# Autodesk Inventor assembly: DarkPoolFacility
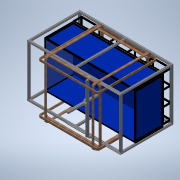
[picture p0: Inventor's stored thumbnail of the model, 180x180]
Saved by Autodesk Inventor 2022 (Build 260153000, 153)
## iProperties
Created: 2021-05-11
Part Number: DarkPoolFacility
Document SubType Name: Assembly
Designer: jamieson-bl
Author: jamieson-bl
## Documents named in this file (9)
- \\Mac\Home\Desktop\WinnipegPMTTestFacility\DarkPoolFacility.iam
- \\Mac\Home\Desktop\WinnipegPMTTestFacility\Room3L10.ipt
- \\Mac\Home\Desktop\WinnipegPMTTestFacility\iManikins\iMan\iMan.iam
- \\Mac\Home\Desktop\WinnipegPMTTestFacility\iManikins\iMandy\iMandy.iam
- \\Mac\Home\Desktop\WinnipegPMTTestFacility\Field Compensation Coils.iam
- \\Mac\Home\Desktop\WinnipegPMTTestFacility\ElectronicsRack.ipt
- \\Mac\Home\Desktop\WinnipegPMTTestFacility\CustomAquariumsStand.ipt
- \\Mac\Home\Desktop\WinnipegPMTTestFacility\CustomAquariumsTank.ipt
- \\Mac\Home\Desktop\WinnipegPMTTestFacility\gantry design\6060gantry.iam
## Components (8 placed, 8 different names)
1. Room3L10:1 — Mate:2, Mate:3
2. iMan:1 [sub-assembly] — Mate:3
3. iMandy:1 [sub-assembly] — Mate:2
4. Field Compensation Coils:1 [sub-assembly] — Mate:5, Mate:6, Mate:7
5. ElectronicsRack:1
6. CustomAquariumsStand:1 — Mate:4, Flush:1, Flush:2, Mate:5, Mate:6, Flush:3, Mate:9
7. CustomAquariumsTank:1 — Mate:4, Flush:1, Flush:2, Mate:7, Mate:8
8. 6060gantry:1 [sub-assembly] — Flush:3, Mate:8, Mate:9
## Relationships (11: Mate 8, Flush 3)
- Mate:2: Room3L10:1 ↔ iMandy:1
- Mate:3: Room3L10:1 ↔ iMan:1
- Mate:4: CustomAquariumsStand:1 ↔ CustomAquariumsTank:1
- Flush:1: CustomAquariumsStand:1 ↔ CustomAquariumsTank:1
- Flush:2: CustomAquariumsStand:1 ↔ CustomAquariumsTank:1
- Mate:5: Field Compensation Coils:1 ↔ CustomAquariumsStand:1
- Mate:6: Field Compensation Coils:1 ↔ CustomAquariumsStand:1
- Mate:7: Field Compensation Coils:1 ↔ CustomAquariumsTank:1
- Flush:3: CustomAquariumsStand:1 ↔ 6060gantry:1
- Mate:8: CustomAquariumsTank:1 ↔ 6060gantry:1
- Mate:9: CustomAquariumsStand:1 ↔ 6060gantry:1
